# Autodesk Inventor assembly: 履带组合范本
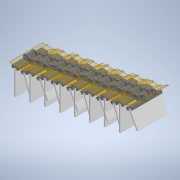
[picture p0: Inventor's stored thumbnail of the model, 180x180]
Saved by Autodesk Inventor 2020 (Build 240168000, 168)
## iProperties
Created: 2019-06-01
Part Number: 履带组合范本
Document SubType Name: Assembly
Designer: aresp
Author: aresp
## Documents named in this file (3)
- D:\vault\ncrCadLib\链轮履带\履带组合范本.iam
- D:\vault\ncrCadLib\链轮履带\高履组合.iam
- D:\vault\ncrCadLib\链轮履带\中履组合.iam
## Components (16 placed, 2 different names)
1. 高履组合:1 [sub-assembly] — 配合:1, 配合:2, 配合:5, 配合:6
2. 中履组合:1 [sub-assembly] — 配合:1, 配合:2
3. 高履组合:2 [sub-assembly] — 配合:13, 配合:14
4. 中履组合:2 [sub-assembly] — 配合:5, 配合:6
5. 高履组合:3 [sub-assembly]
6. 中履组合:3 [sub-assembly] — 配合:13, 配合:14
7. 高履组合:4 [sub-assembly] — 配合:29, 配合:30
8. 中履组合:4 [sub-assembly]
9. 高履组合:5 [sub-assembly]
10. 中履组合:5 [sub-assembly] — 配合:29, 配合:30
11. 高履组合:6 [sub-assembly]
12. 中履组合:6 [sub-assembly]
13. 高履组合:7 [sub-assembly]
14. 中履组合:7 [sub-assembly]
15. 高履组合:8 [sub-assembly]
16. 中履组合:8 [sub-assembly]
## Relationships (30: Mate 30)
- 配合:1 [Mate]: 高履组合:1 ↔ 中履组合:1
- 配合:2 [Mate] (0.1016 mm): 高履组合:1 ↔ 中履组合:1
- [Mate]: 高履组合:2 ↔ 中履组合:2
- [Mate] (0.1016 mm): 高履组合:2 ↔ 中履组合:2
- 配合:5 [Mate]: 高履组合:1 ↔ 中履组合:2
- 配合:6 [Mate]: 高履组合:1 ↔ 中履组合:2
- [Mate]: 高履组合:3 ↔ 中履组合:3
- [Mate] (0.1016 mm): 高履组合:3 ↔ 中履组合:3
- [Mate]: 高履组合:4 ↔ 中履组合:4
- [Mate] (0.1016 mm): 高履组合:4 ↔ 中履组合:4
- [Mate]: 高履组合:3 ↔ 中履组合:4
- [Mate]: 高履组合:3 ↔ 中履组合:4
- 配合:13 [Mate]: 高履组合:2 ↔ 中履组合:3
- 配合:14 [Mate]: 高履组合:2 ↔ 中履组合:3
- [Mate]: 高履组合:5 ↔ 中履组合:5
- [Mate] (0.1016 mm): 高履组合:5 ↔ 中履组合:5
- [Mate]: 高履组合:6 ↔ 中履组合:6
- [Mate] (0.1016 mm): 高履组合:6 ↔ 中履组合:6
- [Mate]: 高履组合:5 ↔ 中履组合:6
- [Mate]: 高履组合:5 ↔ 中履组合:6
- [Mate]: 高履组合:7 ↔ 中履组合:7
- [Mate] (0.1016 mm): 高履组合:7 ↔ 中履组合:7
- [Mate]: 高履组合:8 ↔ 中履组合:8
- [Mate] (0.1016 mm): 高履组合:8 ↔ 中履组合:8
- [Mate]: 高履组合:7 ↔ 中履组合:8
- [Mate]: 高履组合:7 ↔ 中履组合:8
- [Mate]: 高履组合:6 ↔ 中履组合:7
- [Mate]: 高履组合:6 ↔ 中履组合:7
- 配合:29 [Mate]: 高履组合:4 ↔ 中履组合:5
- 配合:30 [Mate]: 高履组合:4 ↔ 中履组合:5
## Named parameters: d2_d1 = 0.1016 mm, d3_d0 = 0 mm, d6_d1 = 0.1016 mm, d7_d2_d1 = 0.1016 mm, d8_d3_d0 = 0 mm, d9_d4 = 0 mm, d10_d5 = 0 mm, d11_d0 = 0 mm, d14_d1 = 0.1016 mm, d15_d2_d1 = 0.1016 mm, d16_d3_d0 = 0 mm, d17_d4 = 0 mm, d18_d5 = 0 mm, d19_d6_d1 = 0.1016 mm, d20_d7_d2_d1 = 0.1016 mm, d21_d8_d3_d0 = 0 mm, d22_d9_d4 = 0 mm, d23_d10_d5 = 0 mm, d24_d11_d0 = 0 mm, d25_d12 = 0 mm, d26_d13 = 0 mm, d27_d0 = 0 mm
